# Autodesk Inventor assembly: base16_assy
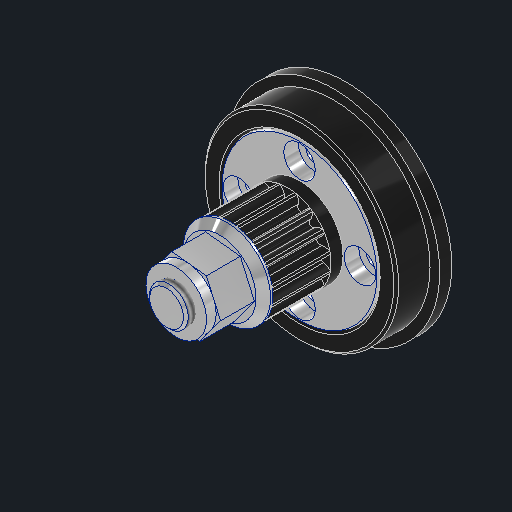
[picture p0: Inventor's stored thumbnail of the model, 512x512]
Saved by Autodesk Inventor 2022 (Build 260153000, 153)
## iProperties
Created: 2021-11-12
Part Number: base16_assy
Document SubType Name: Assembly
Designer: Yuta Kage
Author: Yuta Kage
## Documents named in this file (7)
- C:\Users\yuta0\Documents\GitHub\catchrobo_hardware\assy-scara\base16_assy.iam
- C:\Users\yuta0\Documents\GitHub\catchrobo_hardware\assy-scara\adapter1.ipt
- C:\Users\yuta0\Documents\GitHub\catchrobo_hardware\assy-scara\GEAHBB1_0-16-12-A-8_b.ipt
- C:\Users\yuta0\Documents\GitHub\catchrobo_hardware\assy-scara\nut.ipt
- C:\Users\yuta0\Documents\GitHub\catchrobo_hardware\assy-scara\base13.ipt
- C:\Users\yuta0\Documents\GitHub\catchrobo_hardware\assy-scara\NLDP8.ipt
- C:\Users\yuta0\Documents\GitHub\catchrobo_hardware\assy-scara\base14.ipt
## Components (6 placed, 6 different names)
1. adapter1:1 — メイト:5, メイト:8, メイト:9, メイト:10, メイト:11, メイト:12, メイト:14, メイト:15, メイト:16
2. GEAHBB1_0-16-12-A-8_b:1 — メイト:6, メイト:13, メイト:14
3. nut:1 — メイト:5, メイト:6
4. base13:1 — メイト:8, メイト:9, メイト:10
5. NLDP8:1 — メイト:11, メイト:12, メイト:13
6. base14:1 — メイト:15, メイト:16
## Relationships (11: Mate 11)
- メイト:5 [Mate]: adapter1:1 ↔ nut:1
- メイト:6 [Mate]: GEAHBB1_0-16-12-A-8_b:1 ↔ nut:1
- メイト:8 [Mate]: adapter1:1 ↔ base13:1
- メイト:9 [Mate]: adapter1:1 ↔ base13:1
- メイト:10 [Mate]: adapter1:1 ↔ base13:1
- メイト:11 [Mate]: adapter1:1 ↔ NLDP8:1
- メイト:12 [Mate]: adapter1:1 ↔ NLDP8:1
- メイト:13 [Mate]: GEAHBB1_0-16-12-A-8_b:1 ↔ NLDP8:1
- メイト:14 [Mate]: adapter1:1 ↔ GEAHBB1_0-16-12-A-8_b:1
- メイト:15 [Mate]: adapter1:1 ↔ base14:1
- メイト:16 [Mate]: adapter1:1 ↔ base14:1
